# Autodesk Inventor assembly: 13042026
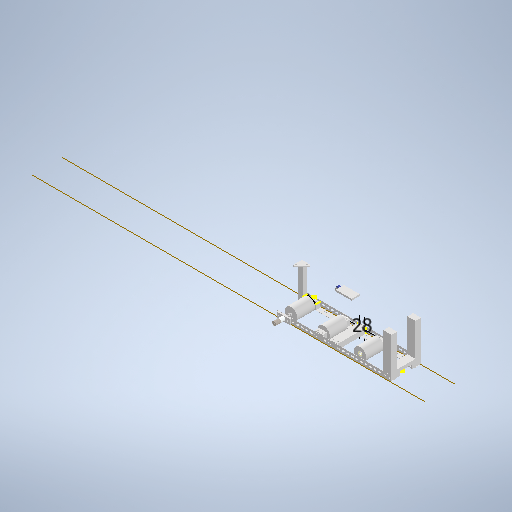
[picture p0: Inventor's stored thumbnail of the model, 512x512]
Saved by Autodesk Inventor 2025.2 (Build 292293000, 293)
## iProperties
Created: 2026-04-13
Part Number: 13042026
Document SubType Name: Assembly
Designer: Oski
Author: Oski
## Documents named in this file (17)
- C:\Users\Oski\Desktop\ProjektPrzejsciowy\Inventor\13042026\13042026.iam
- C:\Users\Oski\Desktop\ProjektPrzejsciowy\Inventor\13042026\Parts\28BYJ48 — kopia\28BYJ48 — kopia\28BYJ48 — kopia.ipt
- C:\Users\Oski\Desktop\ProjektPrzejsciowy\Inventor\13042026\Parts\13042025-02.ipt
- C:\Users\Oski\Desktop\ProjektPrzejsciowy\Inventor\13042026\Parts\706-2_6200ZZ_10x30x9mm_Groove_Ball_Bearing_STEP242\706-2_6200ZZ_10x30x9mm_Groove_Ball_Bearing_STEP242\706-2_6200ZZ_10x30x9mm_Groove_Ball_Bearing_.iam
- C:\Users\Oski\Desktop\ProjektPrzejsciowy\Inventor\13042026\Parts\706-2_6200ZZ_10x30x9mm_Groove_Ball_Bearing_STEP242\25d-metal-gearmotor-172-227\25d-metal-gearmotor-172-227\25d-metal-gearmotor-172-227.ipt
- C:\Users\Oski\Desktop\ProjektPrzejsciowy\Inventor\13042026\Parts\13042026-01.ipt
- C:\Users\Oski\Desktop\ProjektPrzejsciowy\Inventor\13042026\Parts\13042026-04.ipt
- C:\Users\Oski\Desktop\ProjektPrzejsciowy\Inventor\13042026\Parts\13042026-03.ipt
- C:\Users\Oski\Desktop\ProjektPrzejsciowy\Inventor\13042026\Parts\13042026-05.ipt
- C:\Users\Oski\Desktop\ProjektPrzejsciowy\Inventor\13042026\Parts\13042026-06.ipt
- C:\Users\Oski\Desktop\ProjektPrzejsciowy\Inventor\13042026\Parts\m8x40_din933.ipt
- C:\Users\Oski\Desktop\ProjektPrzejsciowy\Inventor\13042026\Parts\1883316.iam
- C:\Users\Oski\Desktop\ProjektPrzejsciowy\Inventor\13042026\Parts\13042026-07.ipt
- C:\Users\Oski\Desktop\ProjektPrzejsciowy\Inventor\13042026\Parts\13042026-09.ipt
- C:\Users\Oski\Desktop\ProjektPrzejsciowy\Inventor\13042026\Parts\13042026-08.ipt
- C:\Users\Oski\Desktop\ProjektPrzejsciowy\Inventor\13042026\Parts\13042026-10.ipt
- C:\Users\Oski\Desktop\ProjektPrzejsciowy\Inventor\13042026\Parts\13042026-11.ipt
## Components (28 placed, 16 different names)
1. 28BYJ48 — kopia:1
2. 13042025-02:1
3. 706-2_6200ZZ_10x30x9mm_Groove_Ball_Bearing_:1 [sub-assembly] — Insert:1, Rotational:2
4. 25d-metal-gearmotor-172-227:1 — Mate:19, Mate:20, Mate:21, Mate:22, Mate:23
5. 13042026-01:1 — Insert:1, Insert:3
6. 13042026-04:1 — Mate:24, Mate:28, Mate:29, Mate:30, Mate:31, Mate:32, Mate:34, Mate:40, Mate:41, Mate:45, Mate:46, Mate:47, Mate:53, Mate:55
7. 13042026-04:2 — Mate:6, Mate:7, Mate:8, Mate:9, Mate:10, Mate:11, Mate:13, Mate:44, Mate:48, Angle:1, Mate:54, Mate:56
8. 13042026-03:1 — Rotational:1, Mate:6, Mate:9, Mate:10, Mate:12, Mate:14
9. 706-2_6200ZZ_10x30x9mm_Groove_Ball_Bearing_:2 [sub-assembly] — Insert:3, Rotational:1
10. 13042026-03:2 — Rotational:2, Mate:34
11. 13042026-06:1 — Mate:7, Mate:8
12. m8x40_din933:1 — Mate:11, Mate:12
13. m8x40_din933:2 — Mate:13, Mate:14
14. 1883316:1 [sub-assembly] — Mate:17, Mate:18
15. 1883316:2 [sub-assembly] — Mate:15, Mate:16
16. 13042026-07:1 — Mate:15, Mate:16, Mate:17, Mate:18, Mate:24, Mate:28, Mate:29
17. 13042026-09:1 — Mate:19, Mate:20, Mate:21, Mate:30, Mate:31, Mate:32
18. 13042026-08:1 — Mate:22, Mate:23, Mate:51, Mate:52
19. 13042026-10:1 — Mate:40, Mate:41, Mate:44
20. 706-2_6200ZZ_10x30x9mm_Groove_Ball_Bearing_:3 [sub-assembly]
21. 13042026-01:2
22. 13042026-03:3 — Mate:45, Mate:46, Mate:47
23. 706-2_6200ZZ_10x30x9mm_Groove_Ball_Bearing_:4 [sub-assembly]
24. 13042026-03:4 — Mate:48
25. 13042026-11:1 — Mate:49, Mate:50, Mate:51, Mate:52, Tangent:1
26. 706-2_6200ZZ_10x30x9mm_Groove_Ball_Bearing_:5 [sub-assembly] — Mate:49, Mate:50
27. 13042026-03:5
28. 13042026-05:1 — Mate:53, Mate:54, Mate:55, Mate:56
## Relationships (51: Mate 40, RevoluteJoint 5, Insert 4, Angle 1, Tangent 1)
- Insert:1: 706-2_6200ZZ_10x30x9mm_Groove_Ball_Bearing_:1 ↔ 13042026-01:1
- Insert:3: 13042026-01:1 ↔ 706-2_6200ZZ_10x30x9mm_Groove_Ball_Bearing_:2
- Rotational:1 [RevoluteJoint]: 13042026-03:1 ↔ 706-2_6200ZZ_10x30x9mm_Groove_Ball_Bearing_:2
- Rotational:2 [RevoluteJoint]: 706-2_6200ZZ_10x30x9mm_Groove_Ball_Bearing_:1 ↔ 13042026-03:2
- Mate:6: 13042026-04:2 ↔ 13042026-03:1
- Mate:7: 13042026-04:2 ↔ 13042026-06:1
- Mate:8: 13042026-04:2 ↔ 13042026-06:1
- Mate:9: 13042026-04:2 ↔ 13042026-03:1
- Mate:10: 13042026-04:2 ↔ 13042026-03:1
- Mate:11: 13042026-04:2 ↔ m8x40_din933:1
- Mate:12: 13042026-03:1 ↔ m8x40_din933:1
- Mate:13: 13042026-04:2 ↔ m8x40_din933:2
- Mate:14: 13042026-03:1 ↔ m8x40_din933:2
- Mate:15: 1883316:2 ↔ 13042026-07:1
- Mate:16: 1883316:2 ↔ 13042026-07:1
- Mate:17: 1883316:1 ↔ 13042026-07:1
- Mate:18: 1883316:1 ↔ 13042026-07:1
- Mate:19: 25d-metal-gearmotor-172-227:1 ↔ 13042026-09:1
- Mate:20: 25d-metal-gearmotor-172-227:1 ↔ 13042026-09:1
- Mate:21: 25d-metal-gearmotor-172-227:1 ↔ 13042026-09:1
- Mate:22: 25d-metal-gearmotor-172-227:1 ↔ 13042026-08:1
- Mate:23: 25d-metal-gearmotor-172-227:1 ↔ 13042026-08:1
- Mate:24: 13042026-04:1 ↔ 13042026-07:1
- Mate:28: 13042026-04:1 ↔ 13042026-07:1
- Mate:29: 13042026-04:1 ↔ 13042026-07:1
- Mate:30: 13042026-04:1 ↔ 13042026-09:1
- Mate:31: 13042026-04:1 ↔ 13042026-09:1
- Mate:32: 13042026-04:1 ↔ 13042026-09:1
- Mate:34: 13042026-04:1 ↔ 13042026-03:2
- Mate:40: 13042026-04:1 ↔ 13042026-10:1
- Mate:41: 13042026-04:1 ↔ 13042026-10:1
- Mate:44: 13042026-04:2 ↔ 13042026-10:1
- [Insert]: 706-2_6200ZZ_10x30x9mm_Groove_Ball_Bearing_:3 ↔ 13042026-01:2
- [Insert]: 13042026-01:2 ↔ 706-2_6200ZZ_10x30x9mm_Groove_Ball_Bearing_:4
- [RevoluteJoint]: 13042026-03:3 ↔ 706-2_6200ZZ_10x30x9mm_Groove_Ball_Bearing_:4
- [RevoluteJoint]: 706-2_6200ZZ_10x30x9mm_Groove_Ball_Bearing_:3 ↔ 13042026-03:4
- Mate:45: 13042026-04:1 ↔ 13042026-03:3
- Mate:46: 13042026-04:1 ↔ 13042026-03:3
- Mate:47: 13042026-04:1 ↔ 13042026-03:3
- Mate:48: 13042026-04:2 ↔ 13042026-03:4
- [RevoluteJoint]: 706-2_6200ZZ_10x30x9mm_Groove_Ball_Bearing_:5 ↔ 13042026-03:5
- Mate:49: 13042026-11:1 ↔ 706-2_6200ZZ_10x30x9mm_Groove_Ball_Bearing_:5
- Mate:50: 13042026-11:1 ↔ 706-2_6200ZZ_10x30x9mm_Groove_Ball_Bearing_:5
- Mate:51: 13042026-08:1 ↔ 13042026-11:1
- Mate:52: 13042026-08:1 ↔ 13042026-11:1
- Angle:1 (0 deg): 13042026-04:2
- Tangent:1: 13042026-11:1
- Mate:53: 13042026-04:1 ↔ 13042026-05:1
- Mate:54: 13042026-04:2 ↔ 13042026-05:1
- Mate:55: 13042026-04:1 ↔ 13042026-05:1
- Mate:56: 13042026-04:2 ↔ 13042026-05:1
## Named parameters: d75_d0 = 0 mm, d76_d2 = 0 mm, d77_d6 = 0 mm, d78_d7 = 63.912393 deg, d79_d8 = 0 mm, d80_d9 = 62.541668 deg, d85_d8 = 0 mm, d86_d9 = -101.748209 deg
